# Autodesk Inventor assembly: Robot Assembly
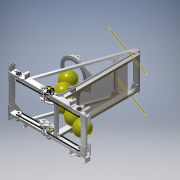
[picture p0: Inventor's stored thumbnail of the model, 180x180]
Saved by Autodesk Inventor 2019.4 (Build 234330000, 330)
## iProperties
Created: 2020-01-06
Part Number: Robot Assembly
Document SubType Name: Assembly
Designer: admin
Author: admin
## Documents named in this file (6)
- C:\Users\Mark\Desktop\7738 Helion Engineering\7738-2020\Robot Assembly.iam
- C:\Users\Mark\Desktop\7738 Helion Engineering\7738-2020\CAD\Drivebase.iam
- C:\Users\Mark\Desktop\7738 Helion Engineering\7738-2020\Intake Mechanism\Intake Mount.ipt
- C:\Users\Mark\Desktop\7738 Helion Engineering\7738-2020\Power Cell.ipt
- C:\Users\Mark\Desktop\7738 Helion Engineering\7738-2020\Turret\Turret Base.iam
- C:\Users\Mark\Desktop\7738 Helion Engineering\7738-2020\Elevator Mechanism\climber.iam
## Components (9 placed, 5 different names)
1. Drivebase:1 [sub-assembly] — Mate:1, Flush:1, Flush:2, Mate:4, Flush:3, Mate:10, Mate:12, Mate:13, Flush:4, Mate:14
2. Intake Mount:1 — Mate:1, Flush:1, Flush:2
3. Power Cell:1 — Mate:5
4. Power Cell:2 — Mate:6
5. Power Cell:3 — Mate:7
6. Power Cell:5 — Mate:9
7. Turret Base:1 [sub-assembly] — Mate:10, Mate:11, Mate:12
8. Power Cell:6
9. climber:1 [sub-assembly] — Mate:13, Flush:4, Mate:14
## Relationships (15: Mate 11, Flush 4)
- Mate:1: Drivebase:1 ↔ Intake Mount:1
- Flush:1: Drivebase:1 ↔ Intake Mount:1
- Flush:2 (130 mm): Drivebase:1 ↔ Intake Mount:1
- Mate:4 (30 mm): Drivebase:1
- Flush:3 (231 mm): Drivebase:1
- Mate:5: Power Cell:1
- Mate:6: Power Cell:2
- Mate:7: Power Cell:3
- Mate:9: Power Cell:5
- Mate:10 (550 mm): Drivebase:1 ↔ Turret Base:1
- Mate:11: Turret Base:1
- Mate:12 (150 mm): Drivebase:1 ↔ Turret Base:1
- Mate:13: Drivebase:1 ↔ climber:1
- Flush:4: Drivebase:1 ↔ climber:1
- Mate:14: Drivebase:1 ↔ climber:1
